# Autodesk Inventor assembly: ThumbDistalPhalanx
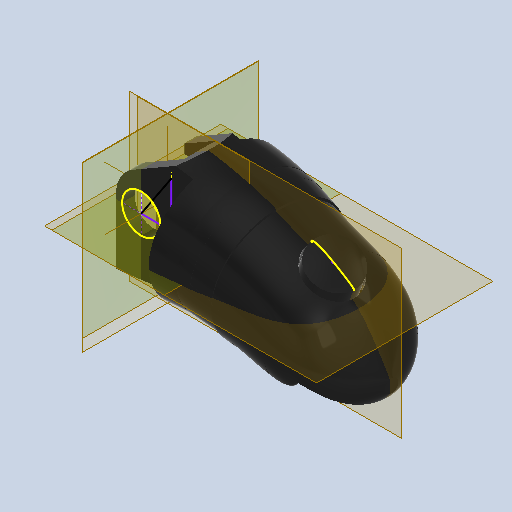
[picture p0: Inventor's stored thumbnail of the model, 512x512]
Saved by Autodesk Inventor 2025.1 (Build 291241000, 241)
## iProperties
Created: 2025-06-05
Part Number: ThumbDistalPhalanx
Document SubType Name: Assembly
Designer: Alexander
Author: Alexander
## Documents named in this file (6)
- D:\Repositorios_Politecnica\TesisProj\Sim Models\ThumbDistalPhalanx.iam
- D:\Repositorios_Politecnica\Handi-EPN\CAD\thumb\DP - D FSR ActuatorTH.ipt
- D:\Repositorios_Politecnica\Handi-EPN\CAD\thumb\DP - D LockTH.ipt
- D:\Repositorios_Politecnica\Handi-EPN\CAD\thumb\DP - D TipTH.ipt
- D:\Repositorios_Politecnica\Handi-EPN\CAD\thumb\DP - D MainTH.ipt
- D:\Repositorios_Politecnica\Handi-EPN\CAD\thumb\DP - P MainTH R.ipt
## Components (5 placed, 5 different names)
1. DP - D FSR ActuatorTH:1 — Mate:1, Mate:2, Mate:4
2. DP - D LockTH:1 — Mate:5, Flush:1, Flush:2, Mate:6, Mate:7, Angle:1
3. DP - D TipTH:1 — Mate:3, Mate:4
4. DP - D MainTH:1 — Mate:1, Mate:2, Mate:3, Mate:5, Flush:1, Flush:2
5. DP - P MainTH R:1 — Mate:6, Mate:7, Angle:1, Mate:8, Mate:9, Flush:3
## Relationships (13: Mate 9, Flush 3, Angle 1)
- Mate:1: DP - D FSR ActuatorTH:1 ↔ DP - D MainTH:1
- Mate:2: DP - D FSR ActuatorTH:1 ↔ DP - D MainTH:1
- Mate:3: DP - D TipTH:1 ↔ DP - D MainTH:1
- Mate:4: DP - D FSR ActuatorTH:1 ↔ DP - D TipTH:1
- Mate:5: DP - D LockTH:1 ↔ DP - D MainTH:1
- Flush:1: DP - D LockTH:1 ↔ DP - D MainTH:1
- Flush:2: DP - D LockTH:1 ↔ DP - D MainTH:1
- Mate:6: DP - D LockTH:1 ↔ DP - P MainTH R:1
- Mate:7: DP - D LockTH:1 ↔ DP - P MainTH R:1
- Angle:1 (180 deg): DP - D LockTH:1 ↔ DP - P MainTH R:1
- Mate:8: DP - P MainTH R:1
- Mate:9: DP - P MainTH R:1
- Flush:3: DP - P MainTH R:1
